# Autodesk Inventor assembly: Micro_Mate-N-Lok_TE-Connectivity_3mm_2x8_Female
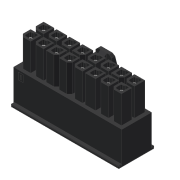
[picture p0: Inventor's stored thumbnail of the model, 180x180]
Saved by Autodesk Inventor 2015 (Build 190159000, 159)
## iProperties
Created: 2015-01-30
Part Number: Micro_Mate-N-Lok_TE-Connectivity_3mm_2x8_Female
Document SubType Name: Assembly
## Documents named in this file (3)
- C:\Dropbox\Inventor\Projects\001_EK-Teile\Micro_Mate-N-Lok_TE-Connectivity_3mm_2x8_Female.iam
- C:\Dropbox\Inventor\Projects\001_EK-Teile\Micro_Mate-N-Lok_TE-Connectivity_3mm_Crimp-Contact_794610-1.ipt
- C:\Dropbox\Inventor\Projects\001_EK-Teile\Micro_Mate-N-Lok_TE-Connectivity_3mm_2x8_Female_1-794617-6.ipt
## Components (17 placed, 2 different names)
1. Micro_Mate-N-Lok_TE-Connectivity_3mm_2x8_Female_1-794617-6:1 — Mate:1, Mate:2, Flush:1
2. Micro_Mate-N-Lok_TE-Connectivity_3mm_Crimp-Contact_794610-1:1 — Mate:1, Mate:2, Flush:1
3. Micro_Mate-N-Lok_TE-Connectivity_3mm_Crimp-Contact_794610-1:2
4. Micro_Mate-N-Lok_TE-Connectivity_3mm_Crimp-Contact_794610-1:3
5. Micro_Mate-N-Lok_TE-Connectivity_3mm_Crimp-Contact_794610-1:4
6. Micro_Mate-N-Lok_TE-Connectivity_3mm_Crimp-Contact_794610-1:5
7. Micro_Mate-N-Lok_TE-Connectivity_3mm_Crimp-Contact_794610-1:6
8. Micro_Mate-N-Lok_TE-Connectivity_3mm_Crimp-Contact_794610-1:7
9. Micro_Mate-N-Lok_TE-Connectivity_3mm_Crimp-Contact_794610-1:8
10. Micro_Mate-N-Lok_TE-Connectivity_3mm_Crimp-Contact_794610-1:9
11. Micro_Mate-N-Lok_TE-Connectivity_3mm_Crimp-Contact_794610-1:10
12. Micro_Mate-N-Lok_TE-Connectivity_3mm_Crimp-Contact_794610-1:11
13. Micro_Mate-N-Lok_TE-Connectivity_3mm_Crimp-Contact_794610-1:12
14. Micro_Mate-N-Lok_TE-Connectivity_3mm_Crimp-Contact_794610-1:13
15. Micro_Mate-N-Lok_TE-Connectivity_3mm_Crimp-Contact_794610-1:14
16. Micro_Mate-N-Lok_TE-Connectivity_3mm_Crimp-Contact_794610-1:15
17. Micro_Mate-N-Lok_TE-Connectivity_3mm_Crimp-Contact_794610-1:16
## Component patterns: (16 elements, first: Micro_Mate-N-Lok_TE-Connectivity_3mm_Crimp-Contact_794610-1:1)
## Relationships (3: Mate 2, Flush 1)
- Mate:1 (0.062 mm): Micro_Mate-N-Lok_TE-Connectivity_3mm_2x8_Female_1-794617-6:1 ↔ Micro_Mate-N-Lok_TE-Connectivity_3mm_Crimp-Contact_794610-1:1
- Mate:2 (0.045 mm): Micro_Mate-N-Lok_TE-Connectivity_3mm_2x8_Female_1-794617-6:1 ↔ Micro_Mate-N-Lok_TE-Connectivity_3mm_Crimp-Contact_794610-1:1
- Flush:1 (-0.1 mm): Micro_Mate-N-Lok_TE-Connectivity_3mm_2x8_Female_1-794617-6:1 ↔ Micro_Mate-N-Lok_TE-Connectivity_3mm_Crimp-Contact_794610-1:1
